# Autodesk Inventor assembly: extension arm assembly horizontal spool
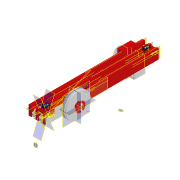
[picture p0: Inventor's stored thumbnail of the model, 180x180]
Saved by Autodesk Inventor 2020 (Build 240168000, 168)
## iProperties
Created: 2020-01-01
Part Number: extension arm assembly horizontal spool
Document SubType Name: Assembly
Designer: ball
Author: ball
## Documents named in this file (11)
- C:\FTC\FTC8863CAD\2019 Robot\Delivery\extension arm\extension arm assembly horizontal spool.iam
- C:\FTC\FTC8863CAD\2019 Robot\Delivery\extension arm\extension arm top.iam
- C:\FTC\FTC8863CAD\2019 Robot\Delivery\extension arm\extension arm middle.iam
- C:\FTC\FTC8863CAD\2019 Robot\Delivery\extension arm\extension arm bottom.iam
- C:\FTC\FTC8863CAD\2019 Robot\Collection\Collector rotator assembly for extension arm.iam
- C:\FTC\FTC8863CAD\2019 Robot\Delivery\Limit switch top + mount left.iam
- C:\FTC\FTC8863CAD\2019 Robot\Delivery\Lift Right\Limit switch top + mount right.iam
- C:\FTC\FTC8863CAD\2019 Robot\Delivery\extension arm\Limit switch trigger spacer extension arm.ipt
- C:\FTC\FTC8863CAD\2019 Robot\Delivery\extension arm\extension arm spool 2_75 with sprocket.iam
- C:\FTC\FTC8863CAD\2019 Robot\Delivery\extension arm\horizontal spool mount bottom.ipt
- C:\FTC\FTC8863CAD\RevRobotics\REV-41-1368 pulley.ipt
## Components (11 placed, 10 different names)
1. extension arm top:1 [sub-assembly] — Mate:1, Mate:3, Mate:4, Mate:5, Mate:17, Mate:18, Mate:19, Mate:26, Mate:27, Flush:1, Flush:4, Flush:6, Mate:29, Mate:33, Mate:35
2. extension arm middle:1 [sub-assembly] — Mate:1, Mate:2, Mate:3, Mate:4, Mate:5, Mate:6, Mate:7, Mate:8, Mate:23, Mate:24, Mate:25
3. extension arm bottom:1 [sub-assembly] — Mate:2, Mate:6, Mate:7, Mate:8, Mate:13, Mate:15, Mate:16
4. Collector rotator assembly for extension arm:1 [sub-assembly] — Mate:13, Mate:15, Mate:16
5. Limit switch top + mount left:1 [sub-assembly] — Mate:17, Mate:18, Mate:19
6. Limit switch top + mount right:1 [sub-assembly] — Mate:26, Mate:27, Flush:1
7. Limit switch trigger spacer extension arm:1 — Mate:23, Mate:24, Mate:25
8. extension arm spool 2_75 with sprocket:1 [sub-assembly] — Mate:28, Flush:6, Mate:29, Flush:7, Flush:8
9. horizontal spool mount bottom:1 — Flush:4, Mate:28, Mate:30, Angle:1, Mate:31, Angle:2
10. REV-41-1368 pulley:1 — Flush:7, Mate:32
11. REV-41-1368 pulley:2 — Flush:8
## Relationships (39: Mate 30, Flush 5, Angle 4)
- Mate:1: extension arm top:1 ↔ extension arm middle:1
- Mate:2: extension arm middle:1 ↔ extension arm bottom:1
- Mate:3: extension arm top:1 ↔ extension arm middle:1
- Mate:4: extension arm top:1 ↔ extension arm middle:1
- Mate:5: extension arm top:1 ↔ extension arm middle:1
- Mate:6: extension arm middle:1 ↔ extension arm bottom:1
- Mate:7: extension arm middle:1 ↔ extension arm bottom:1
- Mate:8: extension arm middle:1 ↔ extension arm bottom:1
- Mate:13: extension arm bottom:1 ↔ Collector rotator assembly for extension arm:1
- Mate:15 (0.254 mm): extension arm bottom:1 ↔ Collector rotator assembly for extension arm:1
- Mate:16: extension arm bottom:1 ↔ Collector rotator assembly for extension arm:1
- Mate:17: extension arm top:1 ↔ Limit switch top + mount left:1
- Mate:18: extension arm top:1 ↔ Limit switch top + mount left:1
- Mate:19: extension arm top:1 ↔ Limit switch top + mount left:1
- Mate:23: extension arm middle:1 ↔ Limit switch trigger spacer extension arm:1
- Mate:24: extension arm middle:1 ↔ Limit switch trigger spacer extension arm:1
- Mate:25: extension arm middle:1 ↔ Limit switch trigger spacer extension arm:1
- Mate:26: extension arm top:1 ↔ Limit switch top + mount right:1
- Mate:27: extension arm top:1 ↔ Limit switch top + mount right:1
- Flush:1: extension arm top:1 ↔ Limit switch top + mount right:1
- Flush:4: extension arm top:1 ↔ horizontal spool mount bottom:1
- Mate:28: extension arm spool 2_75 with sprocket:1 ↔ horizontal spool mount bottom:1
- Flush:6: extension arm top:1 ↔ extension arm spool 2_75 with sprocket:1
- Mate:29 (-88.9 mm): extension arm top:1 ↔ extension arm spool 2_75 with sprocket:1
- Flush:7: extension arm spool 2_75 with sprocket:1 ↔ REV-41-1368 pulley:1
- Flush:8: extension arm spool 2_75 with sprocket:1 ↔ REV-41-1368 pulley:2
- Mate:30: horizontal spool mount bottom:1
- Angle:1 (90 deg): horizontal spool mount bottom:1
- Mate:31: horizontal spool mount bottom:1
- Angle:2 (90 deg): horizontal spool mount bottom:1
- Mate:32: REV-41-1368 pulley:1
- Mate:33: extension arm top:1
- Mate:34
- Mate:35: extension arm top:1
- Mate:36
- Mate:37
- Angle:3 (90 deg)
- Mate:38
- Angle:4 (90 deg)
